# Autodesk Inventor assembly: Door_assembly_v01
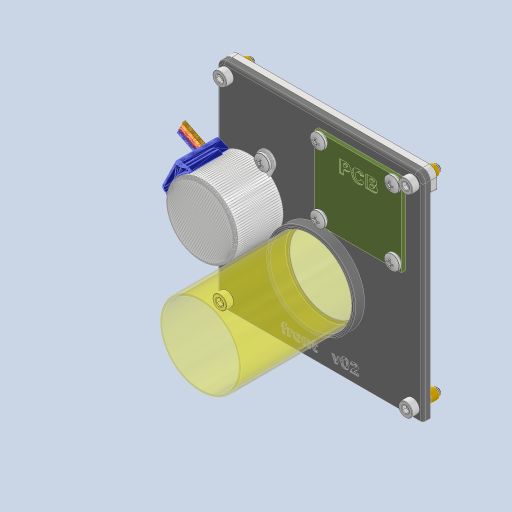
[picture p0: Inventor's stored thumbnail of the model, 512x512]
Saved by Autodesk Inventor 2024.4 (Build 284460000, 460)
## iProperties
Created: 2026-07-13
Part Number: Door_assembly_v01
Document SubType Name: Assembly
Designer: tooles01
Author: tooles01
## iProperties of the stored document MemberDocs/xMigmwfsaOstqfp5jZhjtzgcm2a
Created: 2026-07-13
Part Number: Door_assembly_v01
Document SubType Name: Assembly
Designer: tooles01
Author: tooles01
## iProperties of the stored document MemberDocs/xMag0ln4zDc51gihaEipb25mq0c
Created: 2026-07-13
Part Number: Door_assembly_v01
Document SubType Name: Assembly
Designer: tooles01
Author: tooles01
## iProperties of the stored document MemberDocs/xUlo0whkyJ0k1lroh5jjhx21cJc
Created: 2026-07-13
Part Number: Door_assembly_v01
Document SubType Name: Assembly
Designer: tooles01
Author: tooles01
## Documents named in this file (30)
- C:\Users\Admin\Dropbox (NYU Langone Health)\Shannon_Dropbox\Mar lab\RFID\CAD\Door\Door_assembly_v01.iam
- C:\Users\Admin\Dropbox (NYU Langone Health)\Shannon_Dropbox\Mar lab\RFID\CAD\lib\tube_5cm.ipt
- C:\Users\Admin\Dropbox (NYU Langone Health)\Shannon_Dropbox\Mar lab\RFID\CAD\Door\door_center_01.ipt
- C:\Users\Admin\Dropbox (NYU Langone Health)\Shannon_Dropbox\Mar lab\RFID\CAD\Door\door_front_02.ipt
- C:\Users\Admin\Dropbox (NYU Langone Health)\Shannon_Dropbox\Mar lab\RFID\CAD\lib\M3 heat-set insert.ipt
- C:\Users\Admin\Dropbox (NYU Langone Health)\Shannon_Dropbox\Mar lab\RFID\CAD\lib\92000A114_M3x0.5_5mm_Passivated 18-8 Stainless Steel Pan Head .ipt
- C:\Users\Admin\Dropbox (NYU Langone Health)\Shannon_Dropbox\Mar lab\RFID\CAD\lib\91292A113_M3x0.5_10mm_18-8 Stainless Steel Socket Head Screw.ipt
- C:\Users\Admin\Dropbox (NYU Langone Health)\Shannon_Dropbox\Mar lab\RFID\CAD\Door\PCB_motor.ipt
- C:\Users\Admin\Dropbox (NYU Langone Health)\Shannon_Dropbox\Mar lab\RFID\CAD\Door\door_back_02.ipt
- C:\Users\Admin\Dropbox (NYU Langone Health)\Shannon_Dropbox\Mar lab\RFID\CAD\lib\motor_axle.ipt
- C:\Users\Admin\Dropbox (NYU Langone Health)\Shannon_Dropbox\Mar lab\RFID\CAD\lib\28byj-48-stepper-motor-v9.ipt
- C:\Users\Admin\Dropbox (NYU Langone Health)\Shannon_Dropbox\Mar lab\RFID\CAD\Door\door_03.ipt
- C:\Users\tooles01\NYU Langone Health Dropbox\Shannon Toole\Shannon_Dropbox\Mar lab\RFID\CAD\lib\tube_5cm.ipt
- C:\Users\tooles01\NYU Langone Health Dropbox\Shannon Toole\Shannon_Dropbox\Mar lab\Door\door_center_01.ipt
- C:\Users\tooles01\NYU Langone Health Dropbox\Shannon Toole\Shannon_Dropbox\Mar lab\Door\door_back_01.ipt
- C:\Users\tooles01\NYU Langone Health Dropbox\Shannon Toole\Shannon_Dropbox\Mar lab\Door\lib\motor_axle.ipt
- C:\Users\tooles01\NYU Langone Health Dropbox\Shannon Toole\Shannon_Dropbox\Mar lab\Door\lib\28byj-48-stepper-motor-v9_noaxle.ipt
- C:\Users\tooles01\NYU Langone Health Dropbox\Shannon Toole\Shannon_Dropbox\Mar lab\Door\door_front_02.ipt
- C:\Users\tooles01\NYU Langone Health Dropbox\Shannon Toole\Shannon_Dropbox\Mar lab\Door\door_02.ipt
- C:\Users\tooles01\NYU Langone Health Dropbox\Shannon Toole\Shannon_Dropbox\Mar lab\RFID\CAD\lib\M3 heat-set insert.ipt
- C:\Users\tooles01\Documents\Inventor\Content Center Files\R2024\en-US\ANSI B18.6.7M(00)\ANSI B18.6.7M - M3x0.5 x 5(4).ipt
- C:\Users\tooles01\Documents\Inventor\Content Center Files\R2024\en-US\ANSI B18.3.1M(1)\ANSI B18.3.1M - M3x0.5 x 10(2).ipt
- C:\Users\tooles01\NYU Langone Health Dropbox\Shannon Toole\Shannon_Dropbox\Mar lab\Door\PCB_motor.ipt
- C:\Users\tooles01\NYU Langone Health Dropbox\Shannon Toole\Shannon_Dropbox\Mar lab\RFID\CAD\Door\door_center_01.ipt
- C:\Users\tooles01\NYU Langone Health Dropbox\Shannon Toole\Shannon_Dropbox\Mar lab\RFID\CAD\Door\door_front_02.ipt
- C:\Users\tooles01\NYU Langone Health Dropbox\Shannon Toole\Shannon_Dropbox\Mar lab\RFID\CAD\Door\PCB_motor.ipt
- C:\Users\tooles01\NYU Langone Health Dropbox\Shannon Toole\Shannon_Dropbox\Mar lab\RFID\CAD\Door\door_back_02.ipt
- C:\Users\tooles01\NYU Langone Health Dropbox\Shannon Toole\Shannon_Dropbox\Mar lab\RFID\CAD\lib\motor_axle.ipt
- C:\Users\tooles01\NYU Langone Health Dropbox\Shannon Toole\Shannon_Dropbox\Mar lab\RFID\CAD\lib\28byj-48-stepper-motor-v9.ipt
- C:\Users\tooles01\NYU Langone Health Dropbox\Shannon Toole\Shannon_Dropbox\Mar lab\RFID\CAD\Door\door_03.ipt
## Components (28 placed, 11 different names)
1. tube_5cm:1 — tube to front:1
2. door_center_01:1 — center to front:1, center to front:2, back to center:1, back to center:2
3. door_03:1 — axle to door:1, axle to door:2, axle to door:3
4. 91292A113_M3x0.5_10mm_18-8 Stainless Steel Socket Head Screw:1 — screw to front (mounting):1
5. 91292A113_M3x0.5_10mm_18-8 Stainless Steel Socket Head Screw:2 — screw to front (mounting):2
6. 91292A113_M3x0.5_10mm_18-8 Stainless Steel Socket Head Screw:3 — screw to front (mounting):3
7. 91292A113_M3x0.5_10mm_18-8 Stainless Steel Socket Head Screw:4 — screw to front (mounting):4
8. door_front_02:1 — tube to front:1, center to front:1, center to front:2, motor to front:1, motor to front:2, PCB to front:1, PCB to front:2, heat-set to front (motor):1, heat-set to front (motor):2, heat-set to front (PCB):1, heat-set to front (PCB):2, heat-set to front (PCB):3, heat-set to front (PCB):4, screw to front (mounting):1, screw to front (mounting):2, screw to front (mounting):3, screw to front (mounting):4
9. 28byj-48-stepper-motor-v9:1 — motor to front:1, motor to front:2, axle to motor:1, screw to motor:1, screw to motor:2
10. motor_axle:1 — axle to motor:1, axle to door:1, axle to door:2, axle to door:3
11. PCB_motor:1 — PCB to front:1, PCB to front:2, screw to PCB:1, screw to PCB:2, screw to PCB:3, screw to PCB:4
12. door_back_02:1 — back to center:1, back to center:2, heat-set to back:1, heat-set to back:2, heat-set to back:3, heat-set to back:4
13. M3 heat-set insert:5 — heat-set to front (motor):1
14. M3 heat-set insert:6 — heat-set to front (motor):2
15. M3 heat-set insert:7 — heat-set to front (PCB):1
16. M3 heat-set insert:8 — heat-set to front (PCB):2
17. M3 heat-set insert:9 — heat-set to front (PCB):3
18. M3 heat-set insert:10 — heat-set to front (PCB):4
19. 92000A114_M3x0.5_5mm_Passivated 18-8 Stainless Steel Pan Head :1 — screw to motor:1
20. 92000A114_M3x0.5_5mm_Passivated 18-8 Stainless Steel Pan Head :2 — screw to motor:2
21. 92000A114_M3x0.5_5mm_Passivated 18-8 Stainless Steel Pan Head :3 — screw to PCB:1
22. 92000A114_M3x0.5_5mm_Passivated 18-8 Stainless Steel Pan Head :4 — screw to PCB:2
23. 92000A114_M3x0.5_5mm_Passivated 18-8 Stainless Steel Pan Head :5 — screw to PCB:3
24. 92000A114_M3x0.5_5mm_Passivated 18-8 Stainless Steel Pan Head :6 — screw to PCB:4
25. M3 heat-set insert:1 — heat-set to back:1
26. M3 heat-set insert:2 — heat-set to back:2
27. M3 heat-set insert:3 — heat-set to back:3
28. M3 heat-set insert:4 — heat-set to back:4
## Relationships (33: Insert 29, RevoluteJoint 1, Mate 1, Flush 1, Tangent 1)
- tube to front:1 [Insert]: tube_5cm:1 ↔ door_front_02:1
- center to front:1 [Insert]: door_center_01:1 ↔ door_front_02:1
- center to front:2 [Insert]: door_center_01:1 ↔ door_front_02:1
- back to center:1 [Insert]: door_center_01:1 ↔ door_back_02:1
- back to center:2 [Insert]: door_center_01:1 ↔ door_back_02:1
- axle to motor:1 [RevoluteJoint]: 28byj-48-stepper-motor-v9:1 ↔ motor_axle:1
- axle to door:1 [Mate]: door_03:1 ↔ motor_axle:1
- axle to door:2 [Flush] (-4.25 mm): door_03:1 ↔ motor_axle:1
- axle to door:3 [Tangent]: door_03:1 ↔ motor_axle:1
- motor to front:1 [Insert]: door_front_02:1 ↔ 28byj-48-stepper-motor-v9:1
- motor to front:2 [Insert]: door_front_02:1 ↔ 28byj-48-stepper-motor-v9:1
- PCB to front:1 [Insert]: door_front_02:1 ↔ PCB_motor:1
- PCB to front:2 [Insert]: door_front_02:1 ↔ PCB_motor:1
- heat-set to back:1 [Insert]: door_back_02:1 ↔ M3 heat-set insert:1
- heat-set to back:2 [Insert]: door_back_02:1 ↔ M3 heat-set insert:2
- heat-set to back:3 [Insert]: door_back_02:1 ↔ M3 heat-set insert:3
- heat-set to back:4 [Insert]: door_back_02:1 ↔ M3 heat-set insert:4
- heat-set to front (motor):1 [Insert]: door_front_02:1 ↔ M3 heat-set insert:5
- heat-set to front (motor):2 [Insert]: door_front_02:1 ↔ M3 heat-set insert:6
- screw to motor:1 [Insert]: 28byj-48-stepper-motor-v9:1 ↔ 92000A114_M3x0.5_5mm_Passivated 18-8 Stainless Steel Pan Head :1
- screw to motor:2 [Insert]: 28byj-48-stepper-motor-v9:1 ↔ 92000A114_M3x0.5_5mm_Passivated 18-8 Stainless Steel Pan Head :2
- heat-set to front (PCB):1 [Insert]: door_front_02:1 ↔ M3 heat-set insert:7
- heat-set to front (PCB):2 [Insert]: door_front_02:1 ↔ M3 heat-set insert:8
- heat-set to front (PCB):3 [Insert]: door_front_02:1 ↔ M3 heat-set insert:9
- heat-set to front (PCB):4 [Insert]: door_front_02:1 ↔ M3 heat-set insert:10
- screw to PCB:1 [Insert]: PCB_motor:1 ↔ 92000A114_M3x0.5_5mm_Passivated 18-8 Stainless Steel Pan Head :3
- screw to PCB:2 [Insert]: PCB_motor:1 ↔ 92000A114_M3x0.5_5mm_Passivated 18-8 Stainless Steel Pan Head :4
- screw to PCB:3 [Insert]: PCB_motor:1 ↔ 92000A114_M3x0.5_5mm_Passivated 18-8 Stainless Steel Pan Head :5
- screw to PCB:4 [Insert]: PCB_motor:1 ↔ 92000A114_M3x0.5_5mm_Passivated 18-8 Stainless Steel Pan Head :6
- screw to front (mounting):1 [Insert]: 91292A113_M3x0.5_10mm_18-8 Stainless Steel Socket Head Screw:1 ↔ door_front_02:1
- screw to front (mounting):2 [Insert]: 91292A113_M3x0.5_10mm_18-8 Stainless Steel Socket Head Screw:2 ↔ door_front_02:1
- screw to front (mounting):3 [Insert]: 91292A113_M3x0.5_10mm_18-8 Stainless Steel Socket Head Screw:3 ↔ door_front_02:1
- screw to front (mounting):4 [Insert]: 91292A113_M3x0.5_10mm_18-8 Stainless Steel Socket Head Screw:4 ↔ door_front_02:1
## Named parameters: motor_finish = 0 deg, motor_start = 90 deg
